# Autodesk Inventor assembly: Camera_Full
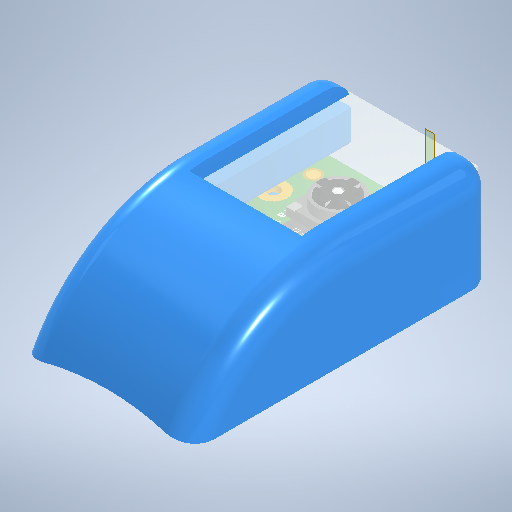
[picture p0: Inventor's stored thumbnail of the model, 512x512]
Saved by Autodesk Inventor 2025.2 (Build 292293000, 293)
## iProperties
Created: 2025-06-17
Part Number: Camera_Full
Document SubType Name: Assembly
Designer: user
Author: user
## Documents named in this file (4)
- E:\nakuu\GLENN\Camera mold\Camera_Full.iam
- E:\nakuu\GLENN\Camera mold\Camera mold\Camera.ipt
- E:\nakuu\GLENN\raspberry-pi-camera-4.snapshot.1\Raspberry pi 3 cam V2,1\Cam V2.1 v1\Cam V2.1 v1\Cam V2.1 v1.ipt
- E:\nakuu\GLENN\Cover.ipt
## Components (3 placed, 3 different names)
1. Camera:1 — Mate:1
2. Cam V2.1 v1:1
3. Cover:1 — Mate:1
## Relationships (1: Mate 1)
- Mate:1: Camera:1 ↔ Cover:1
